# Autodesk Inventor assembly: x_assembly
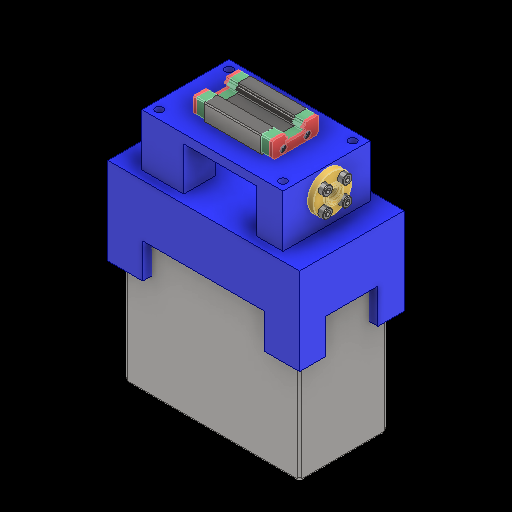
[picture p0: Inventor's stored thumbnail of the model, 512x512]
Saved by Autodesk Inventor 2026.1 (Build 301233000, 233)
## iProperties
Created: 2025-09-28
Part Number: x_assembly
Document SubType Name: Assembly
Designer: drago
Mass: 6775.14 g
Surface Area: 4227.64 cm^2
Volume: 1418.33 cm^3
Density: 4.77685 g/cm^3
Author: drago
## Documents named in this file (11)
- C:\Users\drago\Desktop\_QIST4500_Multidisciplinary_Team_Project\Proteox MX magnet positioner CAD\x_assembly\magnet_assembly.iam
- C:\Users\drago\Desktop\_QIST4500_Multidisciplinary_Team_Project\Proteox MX magnet positioner CAD\x_assembly\y_rail_guide_block.ipt
- C:\Users\drago\Desktop\_QIST4500_Multidisciplinary_Team_Project\Proteox MX magnet positioner CAD\other_parts\Trapezoidal lead screw Nut tr8x8-4.ipt
- C:\Users\drago\Desktop\_QIST4500_Multidisciplinary_Team_Project\Proteox MX magnet positioner CAD\x_assembly\magnet_holder.ipt
- C:\Users\drago\Desktop\_QIST4500_Multidisciplinary_Team_Project\Proteox MX magnet positioner CAD\magnet.ipt
- C:\Users\drago\Documents\Inventor\Content Center Files\R2026\en-US\ISO 4032(2)\ISO 4032 - M3 - ISO.ipt
- C:\Users\drago\Documents\Inventor\Content Center Files\R2026\en-US\ISO 7089\ISO 7089 - 3 - 140 HV(1).ipt
- C:\Users\drago\Desktop\_QIST4500_Multidisciplinary_Team_Project\Proteox MX magnet positioner CAD\x_assembly\magnet_slider_bracket.ipt
- C:\Users\drago\Documents\Inventor\Content Center Files\R2026\en-US\ISO 4762(2)\ISO 4762 - M3 x 10ISO.ipt
- C:\Users\drago\Documents\Inventor\Content Center Files\R2026\en-US\ISO 4762(2)\ISO 4762 - M3 x 25ISO.ipt
- C:\Users\drago\Documents\Inventor\Content Center Files\R2026\en-US\ISO 4762(2)\ISO 4762 - M3 x 16ISO.ipt
## Components (25 placed, 10 different names)
1. y_rail_guide_block:1 — Mate:238, Mate:239, Mate:265
2. Trapezoidal lead screw Nut tr8x8-4:2 — Mate:235, Mate:236, Mate:237, Mate:252, Mate:256, Mate:260, Mate:262
3. magnet:1 — Mate:68, Angle:2, Mate:69, Mate:263, Mate:264
4. magnet_holder:1 — Mate:68, Angle:2, Mate:69, Mate:240, Mate:241, Mate:242, Mate:266, Mate:267, Mate:268, Mate:269, Mate:270, Mate:271, Mate:272, Mate:273
5. magnet_slider_bracket:1 — Mate:235, Mate:236, Mate:237, Mate:238, Mate:239, Mate:240, Mate:241, Mate:242, Mate:243, Mate:244, Mate:245, Mate:246, Mate:247, Mate:248, Mate:249, Mate:250, Mate:251, Mate:253, Mate:254, Mate:255, Mate:257, Mate:258, Mate:259, Mate:261, Mate:265
6. ISO 4762 M3 x 16:1 — Mate:266, Mate:267
7. ISO 4762 M3 x 16:2 — Mate:268, Mate:269
8. ISO 4762 M3 x 16:3 — Mate:270, Mate:271
9. ISO 4762 M3 x 16:4 — Mate:272, Mate:273
10. ISO 7089 3:11 — Mate:243, Mate:244, Insert:19
11. ISO 4762 M3 x 10:1 — Insert:19
12. ISO 7089 3:12 — Mate:245, Mate:246, Insert:20
13. ISO 4762 M3 x 10:2 — Insert:20
14. ISO 7089 3:13 — Mate:247, Mate:248, Insert:21
15. ISO 4762 M3 x 10:3 — Insert:21
16. ISO 7089 3:14 — Mate:249, Mate:250, Insert:22
17. ISO 4762 M3 x 10:4 — Insert:22
18. ISO 4762 M3 x 25:1 — Mate:251, Mate:252
19. ISO 7089 3:15 — Mate:253, Mate:254, Insert:23
20. ISO 4032 M3:16 — Insert:23
21. ISO 4762 M3 x 25:2 — Mate:255, Mate:256
22. ISO 7089 3:16 — Mate:257, Mate:258, Insert:24
23. ISO 4032 M3:17 — Insert:24
24. ISO 4762 M3 x 10:5 — Mate:259, Mate:260
25. ISO 4762 M3 x 10:6 — Mate:261, Mate:262
## Relationships (48: Mate 41, Insert 6, Angle 1)
- Mate:68: magnet:1 ↔ magnet_holder:1
- Angle:2 (0 deg): magnet:1 ↔ magnet_holder:1
- Mate:69: magnet:1 ↔ magnet_holder:1
- Mate:235: Trapezoidal lead screw Nut tr8x8-4:2 ↔ magnet_slider_bracket:1
- Mate:236: Trapezoidal lead screw Nut tr8x8-4:2 ↔ magnet_slider_bracket:1
- Mate:237: Trapezoidal lead screw Nut tr8x8-4:2 ↔ magnet_slider_bracket:1
- Mate:238: y_rail_guide_block:1 ↔ magnet_slider_bracket:1
- Mate:239: y_rail_guide_block:1 ↔ magnet_slider_bracket:1
- Mate:240: magnet_holder:1 ↔ magnet_slider_bracket:1
- Mate:241: magnet_holder:1 ↔ magnet_slider_bracket:1
- Mate:242: magnet_holder:1 ↔ magnet_slider_bracket:1
- Mate:243: magnet_slider_bracket:1 ↔ ISO 7089 3:11
- Mate:244: magnet_slider_bracket:1 ↔ ISO 7089 3:11
- Insert:19: ISO 7089 3:11 ↔ ISO 4762 M3 x 10:1
- Mate:245: magnet_slider_bracket:1 ↔ ISO 7089 3:12
- Mate:246: magnet_slider_bracket:1 ↔ ISO 7089 3:12
- Insert:20: ISO 7089 3:12 ↔ ISO 4762 M3 x 10:2
- Mate:247: magnet_slider_bracket:1 ↔ ISO 7089 3:13
- Mate:248: magnet_slider_bracket:1 ↔ ISO 7089 3:13
- Insert:21: ISO 7089 3:13 ↔ ISO 4762 M3 x 10:3
- Mate:249: magnet_slider_bracket:1 ↔ ISO 7089 3:14
- Mate:250: magnet_slider_bracket:1 ↔ ISO 7089 3:14
- Insert:22: ISO 7089 3:14 ↔ ISO 4762 M3 x 10:4
- Mate:251: magnet_slider_bracket:1 ↔ ISO 4762 M3 x 25:1
- Mate:252: Trapezoidal lead screw Nut tr8x8-4:2 ↔ ISO 4762 M3 x 25:1
- Mate:253: magnet_slider_bracket:1 ↔ ISO 7089 3:15
- Mate:254: magnet_slider_bracket:1 ↔ ISO 7089 3:15
- Insert:23: ISO 7089 3:15 ↔ ISO 4032 M3:16
- Mate:255: magnet_slider_bracket:1 ↔ ISO 4762 M3 x 25:2
- Mate:256: Trapezoidal lead screw Nut tr8x8-4:2 ↔ ISO 4762 M3 x 25:2
- Mate:257: magnet_slider_bracket:1 ↔ ISO 7089 3:16
- Mate:258: magnet_slider_bracket:1 ↔ ISO 7089 3:16
- Insert:24: ISO 7089 3:16 ↔ ISO 4032 M3:17
- Mate:259: magnet_slider_bracket:1 ↔ ISO 4762 M3 x 10:5
- Mate:260: Trapezoidal lead screw Nut tr8x8-4:2 ↔ ISO 4762 M3 x 10:5
- Mate:261: magnet_slider_bracket:1 ↔ ISO 4762 M3 x 10:6
- Mate:262: Trapezoidal lead screw Nut tr8x8-4:2 ↔ ISO 4762 M3 x 10:6
- Mate:263: magnet:1
- Mate:264: magnet:1
- Mate:265: y_rail_guide_block:1 ↔ magnet_slider_bracket:1
- Mate:266: magnet_holder:1 ↔ ISO 4762 M3 x 16:1
- Mate:267: magnet_holder:1 ↔ ISO 4762 M3 x 16:1
- Mate:268: magnet_holder:1 ↔ ISO 4762 M3 x 16:2
- Mate:269: magnet_holder:1 ↔ ISO 4762 M3 x 16:2
- Mate:270: magnet_holder:1 ↔ ISO 4762 M3 x 16:3
- Mate:271: magnet_holder:1 ↔ ISO 4762 M3 x 16:3
- Mate:272: magnet_holder:1 ↔ ISO 4762 M3 x 16:4
- Mate:273: magnet_holder:1 ↔ ISO 4762 M3 x 16:4
